# Autodesk Inventor assembly: Claw
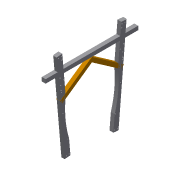
[picture p0: Inventor's stored thumbnail of the model, 180x180]
Saved by Autodesk Inventor 2015 (Build 190159000, 159)
## iProperties
Created: 2015-01-13
Part Number: Claw
Document SubType Name: Assembly
Designer: Collin_2
Author: Collin_2
## Documents named in this file (5)
- C:\Users\Tanner\Desktop\2015 Robot CAD\Devices\Claw\Claw.iam
- C:\Users\Tanner\Desktop\2015 Robot CAD\Devices\Claw\Claw - Base.ipt
- C:\Users\Tanner\Desktop\2015 Robot CAD\Devices\Claw\Yarm.ipt
- C:\Users\Tanner\Desktop\2015 Robot CAD\Devices\Claw\Claw - Arm - Bottom (R) Bottom.ipt
- C:\Users\Tanner\Desktop\2015 Robot CAD\Devices\Claw\Claw - Arm - Top (R) Bottom.ipt
## Components (5 placed, 4 different names)
1. Yarm:1 — Flush:1, Flush:2, Flush:4, Mate:1, Mate:3, Mate:5, Mate:7, Angle:3
2. Yarm:2 — Flush:1, Flush:3, Mate:2, Mate:4, Mate:5, Mate:6, Angle:4, Mate:8
3. Claw - Base:2 — Flush:4, Mate:1, Mate:2, Angle:1, Angle:2, Angle:3, Angle:4, Mate:8
4. Claw - Arm - Bottom (R) Bottom:1 — Flush:2, Mate:3, Angle:2, Mate:7
5. Claw - Arm - Top (R) Bottom:1 — Flush:3, Mate:4, Angle:1, Mate:6
## Relationships (16: Mate 8, Flush 4, Angle 4)
- Flush:1: Yarm:1 ↔ Yarm:2
- Flush:2: Yarm:1 ↔ Claw - Arm - Bottom (R) Bottom:1
- Flush:3: Yarm:2 ↔ Claw - Arm - Top (R) Bottom:1
- Flush:4: Yarm:1 ↔ Claw - Base:2
- Mate:1: Yarm:1 ↔ Claw - Base:2
- Mate:2: Yarm:2 ↔ Claw - Base:2
- Mate:3: Yarm:1 ↔ Claw - Arm - Bottom (R) Bottom:1
- Mate:4: Yarm:2 ↔ Claw - Arm - Top (R) Bottom:1
- Mate:5: Yarm:1 ↔ Yarm:2
- Angle:1 (5 deg): Claw - Base:2 ↔ Claw - Arm - Top (R) Bottom:1
- Angle:2 (-5 deg): Claw - Base:2 ↔ Claw - Arm - Bottom (R) Bottom:1
- Mate:6: Yarm:2 ↔ Claw - Arm - Top (R) Bottom:1
- Mate:7: Yarm:1 ↔ Claw - Arm - Bottom (R) Bottom:1
- Angle:3 (215 deg): Yarm:1 ↔ Claw - Base:2
- Angle:4 (215 deg): Yarm:2 ↔ Claw - Base:2
- Mate:8 (-94.5515 mm): Yarm:2 ↔ Claw - Base:2
